# Autodesk Inventor assembly: ASY-PRS-DRS 940_1200
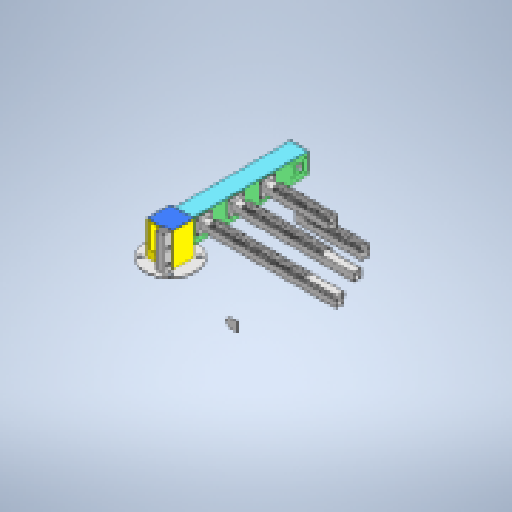
[picture p0: Inventor's stored thumbnail of the model, 512x512]
Saved by Autodesk Inventor 2026.2 (Build 302298000, 298)
## iProperties
Created: 2026-05-12
Part Number: ASY-PRS-DRS 940_1200
Document SubType Name: Assembly
Designer: admin
Author: admin
## Documents named in this file (20)
- C:\Users\admin\Documents\Inventor\PRS-Purovsk\DRS 940\ASY-PRS-DRS 940_1200.iam
- C:\Users\admin\Documents\Inventor\PRS-Purovsk\PRS-1651 FDS MAIN  FLANGE_1200.ipt
- C:\Users\admin\Documents\Inventor\PRS-Purovsk\PRS-169859 DIM filter-distribution-system 1000_1200.ipt
- C:\Users\admin\Documents\Inventor\PRS-Purovsk\PRS-1425 FDS Way FLANGE_1200.ipt
- C:\Users\admin\Documents\Inventor\PRS-Purovsk\ANP 1401 DSB DIMentions_1200.ipt
- C:\Users\admin\Documents\Inventor\PRS-Purovsk\PRS-1662 FDS 1000 way tube 4_1200.ipt
- C:\Users\admin\Documents\Inventor\PRS-Purovsk\PRS-1652 FDS Central tube wall_1200.ipt
- C:\Users\admin\Documents\Inventor\PRS-Purovsk\PRS-1662 FDS 1000 way tube 2_1200.ipt
- C:\Users\admin\Documents\Inventor\PRS-Purovsk\PRS-1663 FDS 1200 way tube 3_1200.ipt
- C:\Users\admin\Documents\Inventor\PRS-Purovsk\PRS-1665 FDS 1000 CUP 1_1200.ipt
- C:\Users\admin\Documents\Inventor\PRS-Purovsk\PRS-1666 FDS 1000 CUP 1_1200.ipt
- C:\Users\admin\Documents\Inventor\PRS-Purovsk\PRS-1422 BOTTOM FDS diameter way up_1200.ipt
- C:\Users\admin\Documents\Inventor\PRS-Purovsk\PRS-1423 BOTTOM FDS diameter way down_1200.ipt
- C:\Users\admin\Documents\Inventor\PRS-Purovsk\PRS-1424 FDS diam way cup_1200.ipt
- C:\Users\admin\Documents\Inventor\PRS-Purovsk\PRS-1661 FDS 1000 way tube 1_1200.ipt
- C:\Users\admin\Documents\Inventor\PRS-Purovsk\PRS-531 roof 1_1200.ipt
- C:\Users\admin\Documents\Inventor\PRS-Purovsk\PRS-532 roof 2_1200.ipt
- C:\Users\admin\Documents\Inventor\PRS-Purovsk\PRS-533 roof 3_1200.ipt
- C:\Users\admin\Documents\Inventor\PRS-Purovsk\PRS-1662 FDS 1000 way tube 4_1200_44.ipt
- C:\Users\admin\Documents\Inventor\PRS-Purovsk\PRS-533 roof 3_1200_44.ipt
## Components (26 placed, 19 different names)
1. PRS-1651 FDS MAIN  FLANGE_1200:1 — Flush:8, Flush:7, Mate:3
2. PRS-169859 DIM filter-distribution-system 1000_1200:1 — Flush:1, Mate:2, Mate:1
3. PRS-1425 FDS Way FLANGE_1200:1 — Rigid:4, Rigid:19
4. ANP 1401 DSB DIMentions_1200:1
5. PRS-1662 FDS 1000 way tube 4_1200:1 — Flush:5, Mate:9, Mate:7, Rigid:21
6. PRS-1652 FDS Central tube wall_1200:1 — Flush:8, Flush:7, Mate:10, Rigid:24, Rigid:22
7. PRS-1652 FDS Central tube wall_1200:2 — Mate:3, Rigid:22
8. PRS-1662 FDS 1000 way tube 2_1200:1 — Mate:8, Flush:6, Mate:6, Rigid:20
9. PRS-1663 FDS 1200 way tube 3_1200:1
10. PRS-1665 FDS 1000 CUP 1_1200:1 — Mate:10
11. PRS-1666 FDS 1000 CUP 1_1200:1
12. PRS-1422 BOTTOM FDS diameter way up_1200:1 — Flush:10, Flush:9, Mate:11, Rigid:23, Rigid:18, Rigid:17, Rigid:16
13. PRS-1423 BOTTOM FDS diameter way down_1200:1 — Rigid:24, Rigid:23, Rigid:4, Rigid:14, Rigid:15, Rigid:13
14. PRS-1424 FDS diam way cup_1200:1 — Flush:10, Flush:9, Mate:11
15. PRS-1425 FDS Way FLANGE_1200:2 — Rigid:20, Rigid:14
16. PRS-1425 FDS Way FLANGE_1200:3 — Rigid:21, Rigid:15
17. PRS-1425 FDS Way FLANGE_1200:4 — Rigid:18
18. PRS-1425 FDS Way FLANGE_1200:5 — Rigid:17
19. PRS-1425 FDS Way FLANGE_1200:6 — Rigid:16
20. PRS-1661 FDS 1000 way tube 1_1200:1 — Mate:5, Mate:4, Flush:4, Rigid:19
21. PRS-531 roof 1_1200:1 — Mate:5, Mate:4, Flush:4
22. PRS-532 roof 2_1200:1 — Mate:8, Flush:6, Mate:6
23. PRS-533 roof 3_1200:1 — Flush:5, Mate:9, Mate:7
24. PRS-1662 FDS 1000 way tube 4_1200_44:1 — Mate:12, Mate:13, Flush:9, Rigid:14
25. PRS-533 roof 3_1200_44:1 — Mate:12, Mate:13, Flush:9
26. PRS-1425 FDS Way FLANGE_1200:7 — Rigid:13, Rigid:14
## Relationships (36: WeldJoint 14, Mate 13, Flush 9)
- Flush:8: PRS-1651 FDS MAIN  FLANGE_1200:1 ↔ PRS-1652 FDS Central tube wall_1200:1
- Flush:7: PRS-1651 FDS MAIN  FLANGE_1200:1 ↔ PRS-1652 FDS Central tube wall_1200:1
- Mate:10: PRS-1652 FDS Central tube wall_1200:1 ↔ PRS-1665 FDS 1000 CUP 1_1200:1
- Flush:1: PRS-169859 DIM filter-distribution-system 1000_1200:1
- Mate:2: PRS-169859 DIM filter-distribution-system 1000_1200:1
- Mate:1: PRS-169859 DIM filter-distribution-system 1000_1200:1
- Flush:10 (1 mm): PRS-1422 BOTTOM FDS diameter way up_1200:1 ↔ PRS-1424 FDS diam way cup_1200:1
- Flush:9 (-1 mm): PRS-1422 BOTTOM FDS diameter way up_1200:1 ↔ PRS-1424 FDS diam way cup_1200:1
- Mate:11: PRS-1422 BOTTOM FDS diameter way up_1200:1 ↔ PRS-1424 FDS diam way cup_1200:1
- Mate:3: PRS-1651 FDS MAIN  FLANGE_1200:1 ↔ PRS-1652 FDS Central tube wall_1200:2
- Mate:5 (10 mm): PRS-1661 FDS 1000 way tube 1_1200:1 ↔ PRS-531 roof 1_1200:1
- Mate:4: PRS-1661 FDS 1000 way tube 1_1200:1 ↔ PRS-531 roof 1_1200:1
- Flush:4 (40 mm): PRS-1661 FDS 1000 way tube 1_1200:1 ↔ PRS-531 roof 1_1200:1
- Mate:8: PRS-1662 FDS 1000 way tube 2_1200:1 ↔ PRS-532 roof 2_1200:1
- Flush:6 (-40 mm): PRS-1662 FDS 1000 way tube 2_1200:1 ↔ PRS-532 roof 2_1200:1
- Mate:6 (10 mm): PRS-1662 FDS 1000 way tube 2_1200:1 ↔ PRS-532 roof 2_1200:1
- Flush:5 (-40 mm): PRS-1662 FDS 1000 way tube 4_1200:1 ↔ PRS-533 roof 3_1200:1
- Mate:9: PRS-1662 FDS 1000 way tube 4_1200:1 ↔ PRS-533 roof 3_1200:1
- Mate:7 (10 mm): PRS-1662 FDS 1000 way tube 4_1200:1 ↔ PRS-533 roof 3_1200:1
- Rigid:24 [WeldJoint]: PRS-1652 FDS Central tube wall_1200:1 ↔ PRS-1423 BOTTOM FDS diameter way down_1200:1
- Rigid:23 [WeldJoint]: PRS-1422 BOTTOM FDS diameter way up_1200:1 ↔ PRS-1423 BOTTOM FDS diameter way down_1200:1
- Rigid:4 [WeldJoint]: PRS-1425 FDS Way FLANGE_1200:1 ↔ PRS-1423 BOTTOM FDS diameter way down_1200:1
- Rigid:22 [WeldJoint]: PRS-1652 FDS Central tube wall_1200:1 ↔ PRS-1652 FDS Central tube wall_1200:2
- Rigid:20 [WeldJoint] (-2 mm): PRS-1662 FDS 1000 way tube 2_1200:1 ↔ PRS-1425 FDS Way FLANGE_1200:2
- Rigid:14 [WeldJoint]: PRS-1423 BOTTOM FDS diameter way down_1200:1 ↔ PRS-1425 FDS Way FLANGE_1200:2
- Rigid:21 [WeldJoint] (-2 mm): PRS-1662 FDS 1000 way tube 4_1200:1 ↔ PRS-1425 FDS Way FLANGE_1200:3
- Rigid:15 [WeldJoint]: PRS-1423 BOTTOM FDS diameter way down_1200:1 ↔ PRS-1425 FDS Way FLANGE_1200:3
- Rigid:18 [WeldJoint]: PRS-1422 BOTTOM FDS diameter way up_1200:1 ↔ PRS-1425 FDS Way FLANGE_1200:4
- Rigid:17 [WeldJoint]: PRS-1422 BOTTOM FDS diameter way up_1200:1 ↔ PRS-1425 FDS Way FLANGE_1200:5
- Rigid:16 [WeldJoint]: PRS-1422 BOTTOM FDS diameter way up_1200:1 ↔ PRS-1425 FDS Way FLANGE_1200:6
- Rigid:19 [WeldJoint] (-2 mm): PRS-1425 FDS Way FLANGE_1200:1 ↔ PRS-1661 FDS 1000 way tube 1_1200:1
- Mate:12 (10 mm): PRS-1662 FDS 1000 way tube 4_1200_44:1 ↔ PRS-533 roof 3_1200_44:1
- Mate:13: PRS-1662 FDS 1000 way tube 4_1200_44:1 ↔ PRS-533 roof 3_1200_44:1
- Flush:9 (-40 mm): PRS-1662 FDS 1000 way tube 4_1200_44:1 ↔ PRS-533 roof 3_1200_44:1
- Rigid:13 [WeldJoint]: PRS-1423 BOTTOM FDS diameter way down_1200:1 ↔ PRS-1425 FDS Way FLANGE_1200:7
- Rigid:14 [WeldJoint]: PRS-1662 FDS 1000 way tube 4_1200_44:1 ↔ PRS-1425 FDS Way FLANGE_1200:7
